# Autodesk Inventor assembly: thumper-bumper-assm-v2
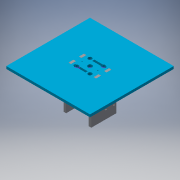
[picture p0: Inventor's stored thumbnail of the model, 180x180]
Saved by Autodesk Inventor 2017 (Build 210142000, 142)
## iProperties
Created: 2017-02-22
Part Number: thumper-bumper-assm-v2
Document SubType Name: Assembly
Designer: John
Author: John
## Documents named in this file (10)
- C:\Users\John\Dropbox\ECE115\pinball-project\thumper-bumper-assm-v2.iam
- C:\Users\John\Dropbox\ECE115\pinball-project\thumper-base-v2.ipt
- C:\Users\John\Dropbox\ECE115\pinball-project\thumper-bumper-sidewall-v2.ipt
- C:\Users\John\Dropbox\ECE115\module-2\Solenoid 1240S\Solenoid.iam
- C:\Users\John\Dropbox\ECE115\pinball-project\game-switch.ipt
- C:\Users\John\Dropbox\ECE115\pinball-project\thumper-bumper-trigger.ipt
- C:\Users\John\Dropbox\ECE115\pinball-project\thumper-bumper-solenoid-interface.ipt
- C:\Users\John\Dropbox\ECE115\pinball-project\thumper-bumper-sidewall3-v2.ipt
- C:\Users\John\Dropbox\ECE115\pinball-project\thumper-bumper-sidewall2-v2.ipt
- C:\Users\John\Dropbox\ECE115\pinball-project\thumper-bumper-top-v2.ipt
## Components (9 placed, 9 different names)
1. thumper-base-v2:1 — Flush:2, Mate:3, Mate:4, Angle:1, Angle:2, Mate:7, Angle:3, Flush:4, Mate:10, Mate:11
2. thumper-bumper-sidewall-v2:2 — Flush:2, Mate:3, Mate:4, Mate:5, Insert:1, Flush:3, Mate:8, Mate:9
3. Solenoid:1 [sub-assembly] — Mate:5, Angle:1, Insert:1, Rotational:1
4. game-switch:1 — Angle:2, Insert:2
5. thumper-bumper-trigger:1 — Mate:7
6. thumper-bumper-solenoid-interface:1 — Rotational:1, Angle:3
7. thumper-bumper-sidewall3-v2:1 — Flush:3, Mate:8, Mate:9, Insert:2
8. thumper-bumper-sidewall2-v2:1 — Flush:4, Mate:10, Mate:11, Flush:5, Mate:12, Mate:13
9. thumper-bumper-top-v2:1 — Flush:5, Mate:12, Mate:13
## Relationships (20: Mate 10, Flush 4, Angle 3, Insert 2, RevoluteJoint 1)
- Flush:2: thumper-base-v2:1 ↔ thumper-bumper-sidewall-v2:2
- Mate:3: thumper-base-v2:1 ↔ thumper-bumper-sidewall-v2:2
- Mate:4: thumper-base-v2:1 ↔ thumper-bumper-sidewall-v2:2
- Mate:5: thumper-bumper-sidewall-v2:2 ↔ Solenoid:1
- Angle:1 (180 deg): thumper-base-v2:1 ↔ Solenoid:1
- Angle:2 (180 deg): thumper-base-v2:1 ↔ game-switch:1
- Mate:7 (1.5 mm): thumper-base-v2:1 ↔ thumper-bumper-trigger:1
- Insert:1: thumper-bumper-sidewall-v2:2 ↔ Solenoid:1
- Rotational:1 [RevoluteJoint]: Solenoid:1 ↔ thumper-bumper-solenoid-interface:1
- Angle:3 (180 deg): thumper-base-v2:1 ↔ thumper-bumper-solenoid-interface:1
- Flush:3: thumper-bumper-sidewall-v2:2 ↔ thumper-bumper-sidewall3-v2:1
- Mate:8: thumper-bumper-sidewall-v2:2 ↔ thumper-bumper-sidewall3-v2:1
- Mate:9: thumper-bumper-sidewall-v2:2 ↔ thumper-bumper-sidewall3-v2:1
- Flush:4: thumper-base-v2:1 ↔ thumper-bumper-sidewall2-v2:1
- Mate:10: thumper-base-v2:1 ↔ thumper-bumper-sidewall2-v2:1
- Mate:11: thumper-base-v2:1 ↔ thumper-bumper-sidewall2-v2:1
- Insert:2: game-switch:1 ↔ thumper-bumper-sidewall3-v2:1
- Flush:5: thumper-bumper-sidewall2-v2:1 ↔ thumper-bumper-top-v2:1
- Mate:12: thumper-bumper-sidewall2-v2:1 ↔ thumper-bumper-top-v2:1
- Mate:13: thumper-bumper-sidewall2-v2:1 ↔ thumper-bumper-top-v2:1
